# Autodesk Inventor assembly: Link2
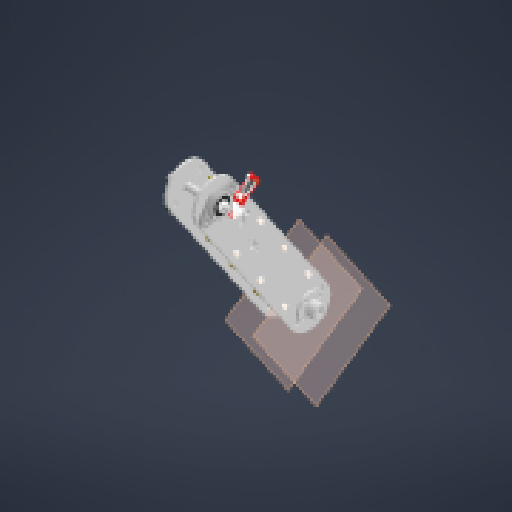
[picture p0: Inventor's stored thumbnail of the model, 512x512]
Saved by Autodesk Inventor 2023 (Build 270158000, 158)
## iProperties
Created: 2023-09-09
Part Number: Link2
Document SubType Name: Assembly
Designer: philo
Author: philo
## Documents named in this file (13)
- C:\Users\philo\OneDrive\Desktop\HK1-2024\TT ROBOT\02_3D_design_new\Link2.iam
- C:\Users\philo\OneDrive\Desktop\HK1-2024\TT ROBOT\02_3D_design_new\Link2Base.ipt
- C:\Users\philo\OneDrive\Desktop\HK1-2024\TT ROBOT\02_3D_design_new\goidoObi.ipt
- C:\Users\philo\OneDrive\Desktop\HK1-2024\TT ROBOT\02_3D_design_new\truc8mm.ipt
- C:\Users\philo\OneDrive\Desktop\HK1-2024\TT ROBOT\02_3D_design_new\GT2 Pulley 20 Tooth (ID6mm).ipt
- C:\Users\philo\OneDrive\Desktop\HK1-2024\TT ROBOT\02_3D_design_new\trudong3mm.ipt
- C:\Users\philo\OneDrive\Desktop\HK1-2024\TT ROBOT\02_3D_design_new\M3 x 5mm.ipt
- C:\Users\philo\OneDrive\Desktop\HK1-2024\TT ROBOT\02_3D_design_new\codinhtruc.ipt
- C:\Users\philo\OneDrive\Desktop\HK1-2024\TT ROBOT\02_3D_design_new\Dongco.iam
- C:\Users\philo\OneDrive\Desktop\HK1-2024\TT ROBOT\02_3D_design_new\limitswitch.ipt
- C:\Users\philo\OneDrive\Desktop\HK1-2024\TT ROBOT\02_3D_design_new\bulong5mmdai50.ipt
- C:\Users\philo\OneDrive\Desktop\HK1-2024\TT ROBOT\02_3D_design_new\oc5mm.ipt
- C:\Users\philo\OneDrive\Desktop\HK1-2024\TT ROBOT\02_3D_design_new\gt2smooth.ipt
## Components (33 placed, 12 different names)
1. limitswitch:2 — Mate:143, Flush:7, Mate:144, Mate:145
2. M3 x 5mm:17 — Mate:129, Mate:136
3. M3 x 5mm:16 — Mate:130, Mate:137
4. M3 x 5mm:15 — Mate:131, Mate:138
5. M3 x 5mm:14 — Mate:132, Mate:139
6. M3 x 5mm:13 — Mate:133, Mate:140
7. M3 x 5mm:12 — Mate:134, Mate:141
8. M3 x 5mm:7 — Mate:118, Mate:119
9. M3 x 5mm:6 — Mate:117, Mate:123
10. M3 x 5mm:5 — Mate:116, Mate:122
11. M3 x 5mm:4 — Mate:115, Mate:121
12. M3 x 5mm:2 — Mate:113, Mate:124
13. M3 x 5mm:1 — Mate:112, Mate:120
14. trudong3mm:9 — Mate:108, Mate:109, Mate:120
15. trudong3mm:8 — Mate:102, Mate:104
16. trudong3mm:7 — Mate:103, Mate:105, Mate:121
17. trudong3mm:3 — Mate:101, Mate:107
18. trudong3mm:2 — Mate:100, Mate:106, Mate:124
19. trudong3mm:1 — Mate:98, Mate:99
20. oc5mm:3 — Mate:96, Mate:97
21. oc5mm:2 — Mate:94, Mate:95
22. gt2smooth:1 — Mate:92, Mate:93
23. oc5mm:1 — Mate:90, Mate:91
24. GT2 Pulley 20 Tooth (ID6mm):1 — Mate:80, Mate:81
25. Dongco:1 [sub-assembly] — Mate:78, Angle:3, Mate:79, Mate:80
26. Link2Base:2 — Mate:71, Mate:72, Mate:73, Mate:74, Mate:75, Angle:2, Mate:78, Mate:79, Mate:81, Mate:88, Flush:6, Mate:89, Mate:90, Mate:93, Mate:98, Mate:99, Mate:100, Mate:101, Mate:102, Mate:103, Mate:104, Mate:105, Mate:106, Mate:107, Mate:108, Mate:109, Mate:129, Mate:130, Mate:131, Mate:132, Mate:133, Mate:134, Mate:136, Mate:137, Mate:138, Mate:139, Mate:140, Mate:141, Mate:143, Flush:7, Mate:144, Mate:145
27. Link2Base:3 — Mate:68, Mate:69, Mate:70, Angle:3, Mate:82, Mate:83, Mate:94, Mate:96, Mate:112, Mate:113, Mate:115, Mate:116, Mate:117, Mate:118, Mate:119, Mate:122, Mate:123
28. goidoObi:2
29. truc8mm:1
30. goidoObi:3 — Mate:74, Mate:75, Angle:2, Mate:82
31. codinhtruc:1 — Mate:68, Mate:69, Mate:70
32. codinhtruc:2 — Mate:71, Mate:72, Mate:73, Mate:83
33. bulong5mmdai50:1 — Mate:88, Flush:6, Mate:89, Mate:91, Mate:92, Mate:95, Mate:97
## Relationships (73: Mate 67, Angle 3, Flush 3)
- [Mate] (30 mm): Link2Base:2 ↔ Link2Base:3
- [Mate]: Link2Base:3 ↔ goidoObi:2
- [Mate]: Link2Base:3 ↔ goidoObi:2
- [Angle] (90 deg): Link2Base:3 ↔ goidoObi:2
- [Flush] (-5 mm): goidoObi:2 ↔ truc8mm:1
- [Mate]: goidoObi:2 ↔ truc8mm:1
- Mate:68: Link2Base:3 ↔ codinhtruc:1
- Mate:69: Link2Base:3 ↔ codinhtruc:1
- Mate:70: Link2Base:3 ↔ codinhtruc:1
- Mate:71: Link2Base:2 ↔ codinhtruc:2
- Mate:72: Link2Base:2 ↔ codinhtruc:2
- Mate:73: Link2Base:2 ↔ codinhtruc:2
- Mate:74: Link2Base:2 ↔ goidoObi:3
- Mate:75: Link2Base:2 ↔ goidoObi:3
- Angle:2 (0 deg): Link2Base:2 ↔ goidoObi:3
- Mate:78: Dongco:1 ↔ Link2Base:2
- Angle:3 (0 deg): Dongco:1 ↔ Link2Base:3
- Mate:79: Dongco:1 ↔ Link2Base:2
- Mate:80: GT2 Pulley 20 Tooth (ID6mm):1 ↔ Dongco:1
- Mate:81 (2 mm): GT2 Pulley 20 Tooth (ID6mm):1 ↔ Link2Base:2
- Mate:82: Link2Base:3 ↔ goidoObi:3
- Mate:83: Link2Base:3 ↔ codinhtruc:2
- Mate:88 (2.5 mm): Link2Base:2 ↔ bulong5mmdai50:1
- Flush:6 (15 mm): Link2Base:2 ↔ bulong5mmdai50:1
- Mate:89: Link2Base:2 ↔ bulong5mmdai50:1
- Mate:90: oc5mm:1 ↔ Link2Base:2
- Mate:91: oc5mm:1 ↔ bulong5mmdai50:1
- Mate:92: gt2smooth:1 ↔ bulong5mmdai50:1
- Mate:93 (8 mm): gt2smooth:1 ↔ Link2Base:2
- Mate:94: oc5mm:2 ↔ Link2Base:3
- Mate:95: oc5mm:2 ↔ bulong5mmdai50:1
- Mate:96: oc5mm:3 ↔ Link2Base:3
- Mate:97: oc5mm:3 ↔ bulong5mmdai50:1
- Mate:98: trudong3mm:1 ↔ Link2Base:2
- Mate:99: trudong3mm:1 ↔ Link2Base:2
- Mate:100: trudong3mm:2 ↔ Link2Base:2
- Mate:101: trudong3mm:3 ↔ Link2Base:2
- Mate:102: trudong3mm:8 ↔ Link2Base:2
- Mate:103: trudong3mm:7 ↔ Link2Base:2
- Mate:104: trudong3mm:8 ↔ Link2Base:2
- Mate:105: trudong3mm:7 ↔ Link2Base:2
- Mate:106: trudong3mm:2 ↔ Link2Base:2
- Mate:107: trudong3mm:3 ↔ Link2Base:2
- Mate:108: trudong3mm:9 ↔ Link2Base:2
- Mate:109: trudong3mm:9 ↔ Link2Base:2
- Mate:112: M3 x 5mm:1 ↔ Link2Base:3
- Mate:113: M3 x 5mm:2 ↔ Link2Base:3
- Mate:115: M3 x 5mm:4 ↔ Link2Base:3
- Mate:116: M3 x 5mm:5 ↔ Link2Base:3
- Mate:117: M3 x 5mm:6 ↔ Link2Base:3
- Mate:118: M3 x 5mm:7 ↔ Link2Base:3
- Mate:119: M3 x 5mm:7 ↔ Link2Base:3
- Mate:120: M3 x 5mm:1 ↔ trudong3mm:9
- Mate:121: M3 x 5mm:4 ↔ trudong3mm:7
- Mate:122: M3 x 5mm:5 ↔ Link2Base:3
- Mate:123: M3 x 5mm:6 ↔ Link2Base:3
- Mate:124: M3 x 5mm:2 ↔ trudong3mm:2
- Mate:129: M3 x 5mm:17 ↔ Link2Base:2
- Mate:130: M3 x 5mm:16 ↔ Link2Base:2
- Mate:131: M3 x 5mm:15 ↔ Link2Base:2
- Mate:132: M3 x 5mm:14 ↔ Link2Base:2
- Mate:133: M3 x 5mm:13 ↔ Link2Base:2
- Mate:134: M3 x 5mm:12 ↔ Link2Base:2
- Mate:136: M3 x 5mm:17 ↔ Link2Base:2
- Mate:137: M3 x 5mm:16 ↔ Link2Base:2
- Mate:138: M3 x 5mm:15 ↔ Link2Base:2
- Mate:139: M3 x 5mm:14 ↔ Link2Base:2
- Mate:140: M3 x 5mm:13 ↔ Link2Base:2
- Mate:141: M3 x 5mm:12 ↔ Link2Base:2
- Mate:143: limitswitch:2 ↔ Link2Base:2
- Flush:7: limitswitch:2 ↔ Link2Base:2
- Mate:144: limitswitch:2 ↔ Link2Base:2
- Mate:145: limitswitch:2 ↔ Link2Base:2
